# Autodesk Inventor assembly: 42146-32
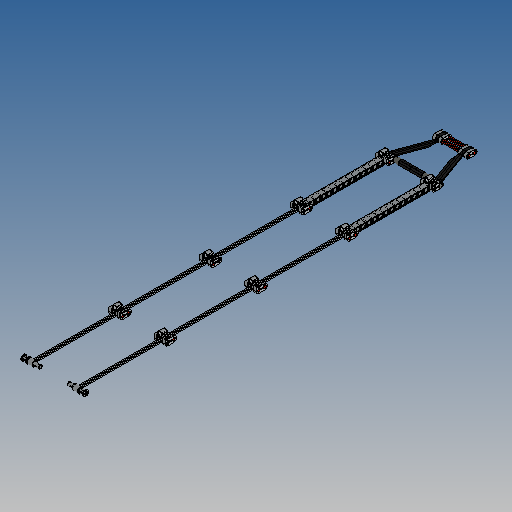
[picture p0: Inventor's stored thumbnail of the model, 512x512]
Saved by Autodesk Inventor 2025 (Build 290162010, 162A)
## iProperties
Created: 2024-12-06
Part Number: 42146-32
Material: Generisch
Document SubType Name: Assembly
Designer: hp.muther
Author: hp.muther
## Documents named in this file (12)
- D:\Inventor\Projekte\Muther\LEGO Technic\LEGO Technik - Raupenkran LR 13000 (42146)\42146-33.iam
- D:\Inventor\Projekte\Muther\LEGO Technic\LEGO Pieces\Verbindungselemente\92907-LtBluishGray.ipt
- D:\Inventor\Projekte\Muther\LEGO Technic\LEGO Pieces\Diverses\32294-Black.ipt
- D:\Inventor\Projekte\Muther\LEGO Technic\LEGO Pieces\Achsen\3706-Red.ipt
- D:\Inventor\Projekte\Muther\LEGO Technic\LEGO Pieces\Achsen\87083-DkBluishGray.ipt
- D:\Inventor\Projekte\Muther\LEGO Technic\LEGO Pieces\Lochbalken schmal\41677-LtBluishGray.ipt
- D:\Inventor\Projekte\Muther\LEGO Technic\LEGO Pieces\Rund\6538c-Black.ipt
- D:\Inventor\Projekte\Muther\LEGO Technic\LEGO Pieces\Lochbalken\32278-LtBluishGray.ipt
- D:\Inventor\Projekte\Muther\LEGO Technic\LEGO Pieces\Achsen\32062-Red.ipt
- D:\Inventor\Projekte\Muther\LEGO Technic\LEGO Pieces\Verbindungselemente\2637-LtBluishGray.ipt
- D:\Inventor\Projekte\Muther\LEGO Technic\LEGO Pieces\Pin's\32054-LtBluishGray.ipt
- D:\Inventor\Projekte\Muther\LEGO Technic\LEGO Pieces\Rund\18654-DkBluishGray.ipt
## Components (47 placed, 11 different names)
1. 92907-LtBluishGray:1 — Einfügen:5, Fluchtend:2, Einfügen:9, Fluchtend:3, Einfügen:17, Einfügen:20
2. 32294-Black:1 — Einfügen:3, Passend:1, Einfügen:4, Einfügen:5
3. 3706-Red:1 — Einfügen:2, Passend:1, Passend:2, Passend:3, Passend:4, Passend:5
4. 3706-Red:2 — Einfügen:1, Einfügen:8
5. 87083-DkBluishGray:1 — Einfügen:9, Einfügen:12
6. 41677-LtBluishGray:1 — Einfügen:4, Passend:2, Fluchtend:2
7. 41677-LtBluishGray:2 — Einfügen:1, Einfügen:2, Einfügen:3
8. 6538c-Black:1 — Einfügen:11, Einfügen:12
9. 32278-LtBluishGray:1 — Einfügen:20, Winkel:1, Einfügen:36
10. 32062-Red:1 — Einfügen:15
11. 32062-Red:2 — Einfügen:17
12. 2637-LtBluishGray:1 — Einfügen:23, Einfügen:27
13. 32054-LtBluishGray:1 — Einfügen:46
14. 32294-Black:2 — Passend:5, Einfügen:10
15. 41677-LtBluishGray:3 — Passend:3
16. 41677-LtBluishGray:4 — Einfügen:8, Passend:4
17. 18654-DkBluishGray:1 — Einfügen:11
18. 92907-LtBluishGray:2 — Einfügen:10, Fluchtend:3, Einfügen:16, Einfügen:18, Einfügen:19
19. 87083-DkBluishGray:2 — Einfügen:14, Einfügen:16
20. 6538c-Black:2 — Einfügen:14, Einfügen:15
21. 18654-DkBluishGray:2
22. 32278-LtBluishGray:2 — Einfügen:19, Winkel:1, Einfügen:35
23. 32062-Red:3 — Einfügen:18
24. 92907-LtBluishGray:3 — Einfügen:22, Einfügen:23, Einfügen:36, Fluchtend:4
25. 32062-Red:4
26. 32062-Red:5 — Einfügen:22
27. 2637-LtBluishGray:2 — Einfügen:43
28. 92907-LtBluishGray:4 — Einfügen:25, Einfügen:27
29. 32062-Red:6
30. 32062-Red:7 — Einfügen:25
31. 2637-LtBluishGray:3 — Einfügen:44
32. 92907-LtBluishGray:5 — Einfügen:29, Einfügen:34
33. 32062-Red:8
34. 32062-Red:9 — Einfügen:29
35. 2637-LtBluishGray:4 — Einfügen:34
36. 92907-LtBluishGray:6 — Einfügen:32, Einfügen:35, Fluchtend:4
37. 32062-Red:10
38. 32062-Red:11 — Einfügen:32
39. 32054-LtBluishGray:2 — Einfügen:45
40. 2637-LtBluishGray:5 — Einfügen:46
41. 92907-LtBluishGray:7 — Einfügen:43
42. 32062-Red:12
43. 32062-Red:13
44. 2637-LtBluishGray:6 — Einfügen:45
45. 92907-LtBluishGray:8 — Einfügen:44
46. 32062-Red:14
47. 32062-Red:15
## Relationships (55: Insert 46, Mate 5, Flush 3, Angle 1)
- Einfügen:1 [Insert]: 3706-Red:2 ↔ 41677-LtBluishGray:2
- Einfügen:2 [Insert]: 3706-Red:1 ↔ 41677-LtBluishGray:2
- Einfügen:3 [Insert]: 32294-Black:1 ↔ 41677-LtBluishGray:2
- Passend:1 [Mate]: 32294-Black:1 ↔ 3706-Red:1
- Einfügen:4 [Insert]: 32294-Black:1 ↔ 41677-LtBluishGray:1
- Passend:2 [Mate]: 3706-Red:1 ↔ 41677-LtBluishGray:1
- Einfügen:5 [Insert]: 92907-LtBluishGray:1 ↔ 32294-Black:1
- Fluchtend:2 [Flush] (-0.4 mm): 92907-LtBluishGray:1 ↔ 41677-LtBluishGray:1
- [Insert]: 32294-Black:2 ↔ 41677-LtBluishGray:4
- [Insert]: 32294-Black:2 ↔ 41677-LtBluishGray:3
- Einfügen:8 [Insert]: 3706-Red:2 ↔ 41677-LtBluishGray:4
- Passend:3 [Mate]: 3706-Red:1 ↔ 41677-LtBluishGray:3
- Passend:4 [Mate]: 3706-Red:1 ↔ 41677-LtBluishGray:4
- Passend:5 [Mate]: 3706-Red:1 ↔ 32294-Black:2
- Einfügen:9 [Insert]: 92907-LtBluishGray:1 ↔ 87083-DkBluishGray:1
- Einfügen:10 [Insert]: 32294-Black:2 ↔ 92907-LtBluishGray:2
- Fluchtend:3 [Flush]: 92907-LtBluishGray:1 ↔ 92907-LtBluishGray:2
- Einfügen:11 [Insert]: 6538c-Black:1 ↔ 18654-DkBluishGray:1
- Einfügen:12 [Insert] (-7.2 mm): 87083-DkBluishGray:1 ↔ 6538c-Black:1
- [Insert]: 6538c-Black:2 ↔ 18654-DkBluishGray:2
- Einfügen:14 [Insert] (-7.2 mm): 87083-DkBluishGray:2 ↔ 6538c-Black:2
- Einfügen:15 [Insert] (-8 mm): 32062-Red:1 ↔ 6538c-Black:2
- Einfügen:16 [Insert]: 92907-LtBluishGray:2 ↔ 87083-DkBluishGray:2
- Einfügen:17 [Insert]: 92907-LtBluishGray:1 ↔ 32062-Red:2
- Einfügen:18 [Insert]: 92907-LtBluishGray:2 ↔ 32062-Red:3
- Einfügen:19 [Insert]: 92907-LtBluishGray:2 ↔ 32278-LtBluishGray:2
- Einfügen:20 [Insert]: 92907-LtBluishGray:1 ↔ 32278-LtBluishGray:1
- Winkel:1 [Angle] (0 deg): 32278-LtBluishGray:1 ↔ 32278-LtBluishGray:2
- [Insert]: 92907-LtBluishGray:3 ↔ 32062-Red:4
- Einfügen:22 [Insert]: 92907-LtBluishGray:3 ↔ 32062-Red:5
- Einfügen:23 [Insert]: 2637-LtBluishGray:1 ↔ 92907-LtBluishGray:3
- [Insert]: 92907-LtBluishGray:4 ↔ 32062-Red:6
- Einfügen:25 [Insert]: 92907-LtBluishGray:4 ↔ 32062-Red:7
- [Insert]: 2637-LtBluishGray:2 ↔ 92907-LtBluishGray:4
- Einfügen:27 [Insert]: 2637-LtBluishGray:1 ↔ 92907-LtBluishGray:4
- [Insert]: 92907-LtBluishGray:5 ↔ 32062-Red:8
- Einfügen:29 [Insert]: 92907-LtBluishGray:5 ↔ 32062-Red:9
- [Insert]: 2637-LtBluishGray:3 ↔ 92907-LtBluishGray:5
- [Insert]: 92907-LtBluishGray:6 ↔ 32062-Red:10
- Einfügen:32 [Insert]: 92907-LtBluishGray:6 ↔ 32062-Red:11
- [Insert]: 2637-LtBluishGray:4 ↔ 92907-LtBluishGray:6
- Einfügen:34 [Insert]: 92907-LtBluishGray:5 ↔ 2637-LtBluishGray:4
- Einfügen:35 [Insert]: 32278-LtBluishGray:2 ↔ 92907-LtBluishGray:6
- Einfügen:36 [Insert]: 32278-LtBluishGray:1 ↔ 92907-LtBluishGray:3
- Fluchtend:4 [Flush]: 92907-LtBluishGray:3 ↔ 92907-LtBluishGray:6
- [Insert]: 92907-LtBluishGray:7 ↔ 32062-Red:12
- [Insert]: 92907-LtBluishGray:7 ↔ 32062-Red:13
- [Insert]: 2637-LtBluishGray:5 ↔ 92907-LtBluishGray:7
- [Insert]: 92907-LtBluishGray:8 ↔ 32062-Red:14
- [Insert]: 92907-LtBluishGray:8 ↔ 32062-Red:15
- [Insert]: 2637-LtBluishGray:6 ↔ 92907-LtBluishGray:8
- Einfügen:43 [Insert]: 2637-LtBluishGray:2 ↔ 92907-LtBluishGray:7
- Einfügen:44 [Insert]: 2637-LtBluishGray:3 ↔ 92907-LtBluishGray:8
- Einfügen:45 [Insert]: 32054-LtBluishGray:2 ↔ 2637-LtBluishGray:6
- Einfügen:46 [Insert]: 32054-LtBluishGray:1 ↔ 2637-LtBluishGray:5
## Named parameters: d9_d2 = 0 mm, d10_d4 = 0 mm, d20_d18 = 0 mm, d21_d19 = -7.2 mm, d29_d24 = 0 mm, d32_d29_d24 = 0 mm, d33_d30 = 0 mm, d34_d31 = 0 mm, d36_d29_d24 = 0 mm, d37_d30 = 0 mm, d38_d31 = 0 mm, d39_d29_d24 = 0 mm, d40_d30 = 0 mm, d41_d31 = 0 mm, d48_d32_d29_d24 = 0 mm, d49_d33_d30 = 0 mm, d50_d34_d31 = 0 mm, d51_d36_d29_d24 = 0 mm, d52_d37_d30 = 0 mm, d53_d38_d31 = 0 mm
